# Autodesk Inventor assembly: chamber_assembly
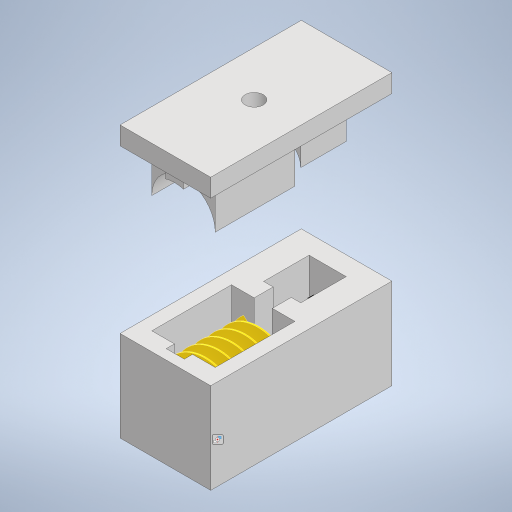
[picture p0: Inventor's stored thumbnail of the model, 512x512]
Saved by Autodesk Inventor 2023 (Build 270158000, 158)
## iProperties
Created: 2023-03-20
Part Number: chamber_assembly
Document SubType Name: Assembly
Designer: caleb
Author: caleb
## Documents named in this file (6)
- C:\Users\caleb\Documents\Inventor\SPICE\chamber_assembly.iam
- C:\Users\caleb\Documents\Inventor\SPICE\dcmotor_housing.ipt
- C:\Users\caleb\Documents\Inventor\SPICE\dcmotor_housing_lid.ipt
- C:\Users\caleb\Documents\Inventor\SPICE\DCMotor.ipt
- C:\Users\caleb\Documents\Inventor\SPICE\DCMotorShaft.ipt
- C:\Users\caleb\Documents\Inventor\SPICE\spiral.ipt
## Components (5 placed, 5 different names)
1. dcmotor_housing:1 — Flush:1, Flush:2, Mate:1, Mate:2, Mate:4, Mate:5
2. dcmotor_housing_lid:1 — Flush:1, Flush:2
3. DCMotor:1 — Rotational:1, Mate:1, Mate:2
4. DCMotorShaft:1 — Rotational:1
5. spiral:1 — Mate:4, Mate:5
## Relationships (7: Mate 4, Flush 2, RevoluteJoint 1)
- Flush:1: dcmotor_housing:1 ↔ dcmotor_housing_lid:1
- Flush:2: dcmotor_housing:1 ↔ dcmotor_housing_lid:1
- Rotational:1 [RevoluteJoint]: DCMotor:1 ↔ DCMotorShaft:1
- Mate:1: dcmotor_housing:1 ↔ DCMotor:1
- Mate:2: dcmotor_housing:1 ↔ DCMotor:1
- Mate:4: dcmotor_housing:1 ↔ spiral:1
- Mate:5: dcmotor_housing:1 ↔ spiral:1
